# Autodesk Inventor assembly: Hip
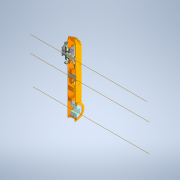
[picture p0: Inventor's stored thumbnail of the model, 180x180]
Saved by Autodesk Inventor 2022.2 (Build 262287030, 287C)
## iProperties
Created: 2022-01-09
Part Number: Hip
Document SubType Name: Assembly
Designer: Jochen
Author: Jochen
## Documents named in this file (10)
- D:\Projects\Lisbeth\CAD\Hip\Hip Short.iam
- D:\Projects\Lisbeth\CAD\Hip\HipBody Short.ipt
- D:\Projects\Lisbeth\CAD\Common\Motor\MotorModule.iam
- D:\Projects\Lisbeth\CAD\Common\Encoder\encoder.iam
- D:\Projects\Lisbeth\CAD\Common\Transmission\TransmissionPulleyCenter.iam
- D:\Projects\Lisbeth\CAD\Common\Transmission\Transmission Pulley.iam
- D:\Projects\Lisbeth\CAD\Common\Belt Tensioner\BeltTensioner 10mm.iam
- D:\Projects\Lisbeth\CAD\Common\Belt Tensioner\MotorBeltTensioner 10mm.iam
- D:\Projects\Lisbeth\CAD\Hip\Hip\Design Accelerator\Synchronous Belts Transmission1.iam
- D:\Projects\Lisbeth\CAD\Hip\Hip\Design Accelerator\Synchronous Belts Transmission2.iam
## Components (9 placed, 8 different names)
1. HipBody:1 — Mate:1, Mate:2, Mate:3, Mate:4, Mate:5, Mate:7, Mate:8, Mate:9, Mate:10, Mate:11, Mate:12, Mate:13, Mate:14
2. MotorModule:2 [sub-assembly] — Mate:1, Mate:2, Mate:13
3. Encoder:2 [sub-assembly] — Mate:3, Mate:4, Angle:1
4. TransmissionPuileyCenter:1 [sub-assembly] — Mate:5, Mate:8
5. Transmission Pulley:1 [sub-assembly] — Mate:7, Mate:14
6. Belt tensioner:1 [sub-assembly] — Mate:9, Mate:10
7. MotorBeltTensioner:1 [sub-assembly] — Mate:11, Mate:12
8. Synchronous Belts Transmission:1 [sub-assembly]
9. Synchronous Belts Transmission:2 [sub-assembly]
## Relationships (14: Mate 13, Angle 1)
- Mate:1: HipBody:1 ↔ MotorModule:2
- Mate:2: HipBody:1 ↔ MotorModule:2
- Mate:3: HipBody:1 ↔ Encoder:2
- Mate:4: HipBody:1 ↔ Encoder:2
- Angle:1 (0 deg): Encoder:2
- Mate:5: HipBody:1 ↔ TransmissionPuileyCenter:1
- Mate:7: HipBody:1 ↔ Transmission Pulley:1
- Mate:8: HipBody:1 ↔ TransmissionPuileyCenter:1
- Mate:9: HipBody:1 ↔ Belt tensioner:1
- Mate:10: HipBody:1 ↔ Belt tensioner:1
- Mate:11: HipBody:1 ↔ MotorBeltTensioner:1
- Mate:12: HipBody:1 ↔ MotorBeltTensioner:1
- Mate:13: HipBody:1 ↔ MotorModule:2
- Mate:14: HipBody:1 ↔ Transmission Pulley:1
